# Autodesk Inventor assembly: camera_rack
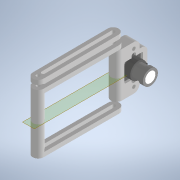
[picture p0: Inventor's stored thumbnail of the model, 180x180]
Saved by Autodesk Inventor 2020 (Build 240168000, 168)
## iProperties
Created: 2022-10-14
Part Number: camera_rack
Document SubType Name: Assembly
Designer: akapu
Author: akapu
## Documents named in this file (5)
- C:\Users\akapu\Documents\maze bot\camera_rack.iam
- C:\Users\akapu\Documents\maze bot\arrow.ipt
- C:\Users\akapu\Documents\maze bot\OpenMV H7\openmv4_h7.iam
- C:\Users\akapu\Documents\maze bot\ramka.ipt
- C:\Users\akapu\Documents\maze bot\holder.ipt
## Components (4 placed, 4 different names)
1. arrow:1 — Совмещение:1
2. openmv4_h7:1 [sub-assembly] — Заподлицо:1
3. ramka:1 — Заподлицо:1, Заподлицо:2, Совмещение:2
4. holder:1 — Совмещение:1, Заподлицо:2, Совмещение:2
## Relationships (4: Flush 2, Mate 2)
- Заподлицо:1 [Flush]: openmv4_h7:1 ↔ ramka:1
- Совмещение:1 [Mate]: arrow:1 ↔ holder:1
- Заподлицо:2 [Flush]: ramka:1 ↔ holder:1
- Совмещение:2 [Mate] (9 mm): ramka:1 ↔ holder:1
